# Autodesk Inventor assembly: BearingTable
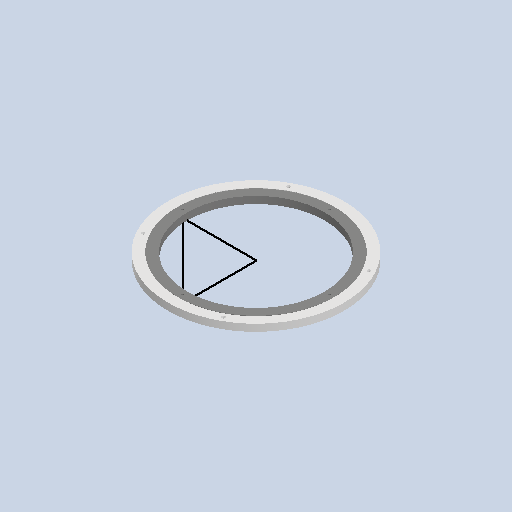
[picture p0: Inventor's stored thumbnail of the model, 512x512]
Saved by Autodesk Inventor 2023 (Build 270158000, 158)
## iProperties
Created: 2023-03-23
Part Number: BearingTable
Document SubType Name: Assembly
Designer: czapa
Author: czapa
## Documents named in this file (3)
- C:\Users\czapa\OneDrive\Documents\GitHub\S.P.I.C.E\3D Models\Version1\BearingTable.iam
- C:\Users\czapa\OneDrive\Documents\GitHub\S.P.I.C.E\3D Models\Version1\InnerBearingTable.ipt
- C:\Users\czapa\OneDrive\Documents\GitHub\S.P.I.C.E\3D Models\Version1\OuterBearingTable.ipt
## Components (2 placed, 2 different names)
1. InnerBearingTable:1 — Mate:1, Flush:1
2. OuterBearingTable:1 — Mate:1, Flush:1
## Relationships (2: Mate 1, Flush 1)
- Mate:1: InnerBearingTable:1 ↔ OuterBearingTable:1
- Flush:1: InnerBearingTable:1 ↔ OuterBearingTable:1
